# Autodesk Inventor assembly: Adamant Cover
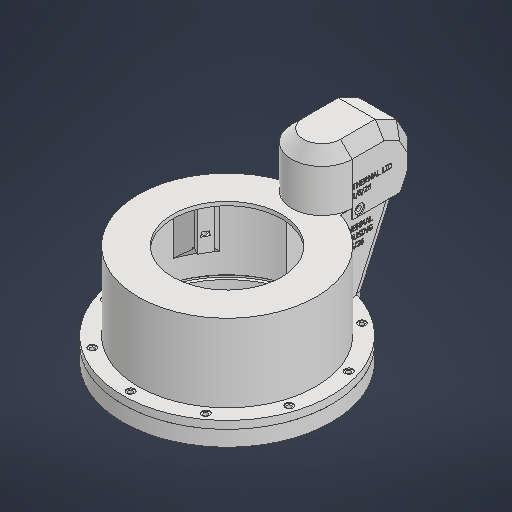
[picture p0: Inventor's stored thumbnail of the model, 512x512]
Saved by Autodesk Inventor 2026.2 (Build 302298000, 298)
## iProperties
Created: 2026-01-05
Part Number: Adamant Cover
Document SubType Name: Assembly
Designer: mumin
Author: mumin
## Documents named in this file (4)
- C:\GitHub\In-situ-monitoring-of-powder-bed-fusion-additive-manufacturing\system_development\Adamant\v0.2\hardware_development\Adamant Cover.iam
- C:\GitHub\In-situ-monitoring-of-powder-bed-fusion-additive-manufacturing\system_development\Adamant\v0.2\hardware_development\Cover parts\New Thermal Housing.ipt
- C:\GitHub\In-situ-monitoring-of-powder-bed-fusion-additive-manufacturing\system_development\Adamant\v0.2\hardware_development\Cover parts\New Thermal Lid.ipt
- C:\GitHub\In-situ-monitoring-of-powder-bed-fusion-additive-manufacturing\system_development\Adamant\v0.2\hardware_development\Cover parts\SealedGlassRing.ipt
## Components (3 placed, 3 different names)
1. New Thermal Housing:1 — Mate:1, Mate:2, Mate:3, Insert:1, Insert:2
2. New Thermal Lid:1 — Mate:1, Mate:2, Mate:3
3. SealedGlassRing:1 — Insert:1, Insert:2
## Relationships (5: Mate 3, Insert 2)
- Mate:1: New Thermal Housing:1 ↔ New Thermal Lid:1
- Mate:2: New Thermal Housing:1 ↔ New Thermal Lid:1
- Mate:3: New Thermal Housing:1 ↔ New Thermal Lid:1
- Insert:1: New Thermal Housing:1 ↔ SealedGlassRing:1
- Insert:2: New Thermal Housing:1 ↔ SealedGlassRing:1
